# Autodesk Inventor assembly: 071_1000_fipt_cell
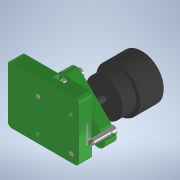
[picture p0: Inventor's stored thumbnail of the model, 180x180]
Saved by Autodesk Inventor 2020 (Build 240168000, 168)
## iProperties
Created: 2020-04-29
Part Number: 071_1000_fipt_cell
Document SubType Name: Assembly
Designer: deniz
Author: deniz
## Documents named in this file (8)
- C:\Repo\fipt_project\fipt\cad\fipt_cell\071_1000_fipt_cell.iam
- C:\Repo\fipt_project\fipt\cad\fipt_cell\071_0100_Base.ipt
- C:\Repo\fipt_project\fipt\cad\fipt_cell\071_0101_Top.ipt
- C:\Repo\fipt_project\fipt\cad\fipt_cell\071_0102_Clamp.ipt
- C:\Repo\fipt_project\fipt\cad\fipt_cell\071_0122_FoamKapton_long.ipt
- C:\Repo\fipt_project\fipt\cad\fipt_cell\071_0121_FoamKapton_short.ipt
- C:\Repo\fipt_project\fipt\cad\fipt_cell\components\Torque limiting knob screw GN 5910-47-M6-30-1-SW.ipt
- C:\Repo\fipt_project\fipt\cad\fipt_cell\components\ISO 4762 - M5 x 40ISO.ipt
## Components (8 placed, 7 different names)
1. 071_0100_Base:1 — Mate:1, Mate:7, Flush:5, Mate:8, Mate:12, Mate:13
2. 071_0101_Top:1 — Mate:6, Flush:3, Flush:4, Mate:12, Mate:13, Mate:15
3. ISO 4762 M5 x 40:1 — Mate:1
4. ISO 4762 M5 x 40:2
5. 071_0102_Clamp:1 — Mate:14
6. 071_0122_FoamKapton_long:1 — Mate:7, Flush:5, Mate:8
7. 071_0121_FoamKapton_short:1 — Mate:6, Flush:3, Flush:4
8. Torque limiting knob screw GN 5910-47-M6-30-1-SW:1 — Mate:14, Mate:15
## Relationships (16: Mate 11, Flush 5)
- [Flush]: 071_0100_Base:1 ↔ ISO 4762 M5 x 40:1
- [Flush]: 071_0100_Base:1 ↔ ISO 4762 M5 x 40:2
- Mate:1: 071_0100_Base:1 ↔ ISO 4762 M5 x 40:1
- [Mate]: 071_0100_Base:1 ↔ ISO 4762 M5 x 40:2
- [Mate]: ISO 4762 M5 x 40:1 ↔ 071_0102_Clamp:1
- [Mate]: ISO 4762 M5 x 40:1 ↔ 071_0102_Clamp:1
- Mate:6: 071_0101_Top:1 ↔ 071_0121_FoamKapton_short:1
- Flush:3: 071_0101_Top:1 ↔ 071_0121_FoamKapton_short:1
- Flush:4: 071_0101_Top:1 ↔ 071_0121_FoamKapton_short:1
- Mate:7: 071_0100_Base:1 ↔ 071_0122_FoamKapton_long:1
- Flush:5: 071_0100_Base:1 ↔ 071_0122_FoamKapton_long:1
- Mate:8: 071_0100_Base:1 ↔ 071_0122_FoamKapton_long:1
- Mate:12 (0.2 mm): 071_0100_Base:1 ↔ 071_0101_Top:1
- Mate:13 (0.2 mm): 071_0100_Base:1 ↔ 071_0101_Top:1
- Mate:14: 071_0102_Clamp:1 ↔ Torque limiting knob screw GN 5910-47-M6-30-1-SW:1
- Mate:15: 071_0101_Top:1 ↔ Torque limiting knob screw GN 5910-47-M6-30-1-SW:1
